# Autodesk Inventor assembly: mobile_robot_car_motor230
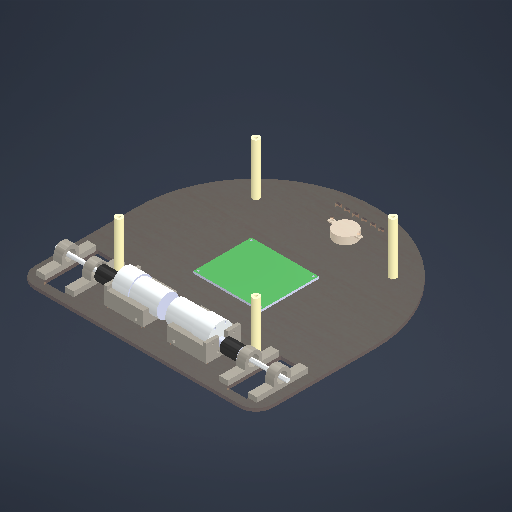
[picture p0: Inventor's stored thumbnail of the model, 512x512]
Saved by Autodesk Inventor 2026 (Build 300175050, 175E)
## iProperties
Created: 2025-06-05
Part Number: mobile_robot_car_motor230
Document SubType Name: Assembly
Designer: satom
Author: satom
## Documents named in this file (11)
- C:\Users\satom\Desktop\Robot\CAD\Inventor\mobile_robot_car_motor230.iam
- C:\Users\satom\Desktop\Robot\CAD\Inventor\C - Chassis\layer1_new_motor2.ipt
- C:\Users\satom\Desktop\Robot\CAD\Inventor\solidworks\D - DriveTrain\motor_FIT0403_122rpm\motor_FIT0403_122rpm\motor_FIT0403_122rpm.ipt
- C:\Users\satom\Desktop\Robot\CAD\Inventor\solidworks\D - DriveTrain\motor_holder_FIT0403_122rpm\motor_holder_FIT0403_122rpm\motor_holder_FIT0403_122rpm.ipt
- C:\Users\satom\Desktop\Robot\CAD\Inventor\solidworks\D - DriveTrain\wheel_bearing_FIT0403_122rpm\wheel_bearing_FIT0403_122rpm\wheel_bearing_FIT0403_122rpm.ipt
- C:\Users\satom\Desktop\Robot\CAD\Inventor\solidworks\D - DriveTrain\wheel_bearing\wheel_bearing\wheel_bearing.ipt
- C:\Users\satom\Desktop\Robot\CAD\Inventor\solidworks\D - DriveTrain\shaft_coupler 6 mm\shaft_coupler 6 mm\shaft_coupler 6 mm.ipt
- C:\Users\satom\Desktop\Robot\CAD\Inventor\solidworks\D - DriveTrain\drive_shaft\drive_shaft\drive_shaft.ipt
- C:\Users\satom\Desktop\Robot\CAD\Inventor\C - Chassis\3inch_standoff.ipt
- C:\Users\satom\Desktop\Robot\CAD\Inventor\solidworks\E - Electronics\Main Board\Main Board\Main Board.ipt
- C:\Users\satom\Desktop\Robot\CAD\Inventor\solidworks\D - DriveTrain\ball_caster\ball_caster\ball_caster.ipt
## Components (19 placed, 10 different names)
1. layer1_new_motor2:1 — Mate:1, Mate:2, Mate:9, Mate:10, Mate:11, Mate:12, Mate:13, Mate:14, Mate:15, Mate:16, Mate:17, Mate:18, Mate:19, Mate:20, Mate:21, Mate:22, Mate:23, Mate:24, Mate:25, Mate:26, Mate:35, Mate:36, Mate:37, Mate:38, Mate:39, Mate:40, Mate:41, Mate:42, Mate:43, Mate:44, Mate:45, Mate:46, Mate:47, Mate:48
2. motor_FIT0403_122rpm:1 — Mate:4, Mate:6, Mate:8, Mate:28, Mate:29
3. motor_FIT0403_122rpm:2 — Mate:3, Mate:5, Mate:7, Mate:27, Mate:30
4. motor_holder_FIT0403_122rpm:1 — Mate:2, Mate:4, Mate:6, Mate:8, Mate:12, Mate:13, Mate:14
5. motor_holder_FIT0403_122rpm:2 — Mate:1, Mate:3, Mate:5, Mate:7, Mate:9, Mate:10, Mate:11
6. wheel_bearing_FIT0403_122rpm:1 — Mate:15, Mate:16, Mate:17
7. wheel_bearing_FIT0403_122rpm:2 — Mate:18, Mate:19, Mate:20
8. wheel_bearing:1 — Mate:21, Mate:25, Mate:26
9. wheel_bearing:2 — Mate:22, Mate:23, Mate:24
10. shaft_coupler 6 mm:1 — Mate:27, Mate:30, Mate:32, Mate:33
11. shaft_coupler 6 mm:2 — Mate:28, Mate:29, Mate:31, Mate:34
12. drive_shaft:1 — Mate:32, Mate:33
13. drive_shaft:2 — Mate:31, Mate:34
14. 3inch_standoff:1 — Mate:36, Mate:37
15. 3inch_standoff:2 — Mate:35, Mate:38
16. Main Board:1 — Mate:39, Mate:40, Mate:41
17. ball_caster:1 — Mate:42, Mate:43, Mate:44
18. 3inch_standoff:3 — Mate:46, Mate:47
19. 3inch_standoff:4 — Mate:45, Mate:48
## Relationships (48: Mate 48)
- Mate:1: layer1_new_motor2:1 ↔ motor_holder_FIT0403_122rpm:2
- Mate:2: layer1_new_motor2:1 ↔ motor_holder_FIT0403_122rpm:1
- Mate:3: motor_FIT0403_122rpm:2 ↔ motor_holder_FIT0403_122rpm:2
- Mate:4: motor_FIT0403_122rpm:1 ↔ motor_holder_FIT0403_122rpm:1
- Mate:5: motor_FIT0403_122rpm:2 ↔ motor_holder_FIT0403_122rpm:2
- Mate:6: motor_FIT0403_122rpm:1 ↔ motor_holder_FIT0403_122rpm:1
- Mate:7: motor_FIT0403_122rpm:2 ↔ motor_holder_FIT0403_122rpm:2
- Mate:8: motor_FIT0403_122rpm:1 ↔ motor_holder_FIT0403_122rpm:1
- Mate:9: layer1_new_motor2:1 ↔ motor_holder_FIT0403_122rpm:2
- Mate:10: layer1_new_motor2:1 ↔ motor_holder_FIT0403_122rpm:2
- Mate:11: layer1_new_motor2:1 ↔ motor_holder_FIT0403_122rpm:2
- Mate:12: layer1_new_motor2:1 ↔ motor_holder_FIT0403_122rpm:1
- Mate:13: layer1_new_motor2:1 ↔ motor_holder_FIT0403_122rpm:1
- Mate:14: layer1_new_motor2:1 ↔ motor_holder_FIT0403_122rpm:1
- Mate:15: layer1_new_motor2:1 ↔ wheel_bearing_FIT0403_122rpm:1
- Mate:16: layer1_new_motor2:1 ↔ wheel_bearing_FIT0403_122rpm:1
- Mate:17: layer1_new_motor2:1 ↔ wheel_bearing_FIT0403_122rpm:1
- Mate:18: layer1_new_motor2:1 ↔ wheel_bearing_FIT0403_122rpm:2
- Mate:19: layer1_new_motor2:1 ↔ wheel_bearing_FIT0403_122rpm:2
- Mate:20: layer1_new_motor2:1 ↔ wheel_bearing_FIT0403_122rpm:2
- Mate:21: layer1_new_motor2:1 ↔ wheel_bearing:1
- Mate:22: layer1_new_motor2:1 ↔ wheel_bearing:2
- Mate:23: layer1_new_motor2:1 ↔ wheel_bearing:2
- Mate:24: layer1_new_motor2:1 ↔ wheel_bearing:2
- Mate:25: layer1_new_motor2:1 ↔ wheel_bearing:1
- Mate:26: layer1_new_motor2:1 ↔ wheel_bearing:1
- Mate:27: motor_FIT0403_122rpm:2 ↔ shaft_coupler 6 mm:1
- Mate:28: motor_FIT0403_122rpm:1 ↔ shaft_coupler 6 mm:2
- Mate:29: motor_FIT0403_122rpm:1 ↔ shaft_coupler 6 mm:2
- Mate:30: motor_FIT0403_122rpm:2 ↔ shaft_coupler 6 mm:1
- Mate:31: shaft_coupler 6 mm:2 ↔ drive_shaft:2
- Mate:32: shaft_coupler 6 mm:1 ↔ drive_shaft:1
- Mate:33: shaft_coupler 6 mm:1 ↔ drive_shaft:1
- Mate:34: shaft_coupler 6 mm:2 ↔ drive_shaft:2
- Mate:35: layer1_new_motor2:1 ↔ 3inch_standoff:2
- Mate:36: layer1_new_motor2:1 ↔ 3inch_standoff:1
- Mate:37: layer1_new_motor2:1 ↔ 3inch_standoff:1
- Mate:38: layer1_new_motor2:1 ↔ 3inch_standoff:2
- Mate:39: layer1_new_motor2:1 ↔ Main Board:1
- Mate:40: layer1_new_motor2:1 ↔ Main Board:1
- Mate:41: layer1_new_motor2:1 ↔ Main Board:1
- Mate:42: layer1_new_motor2:1 ↔ ball_caster:1
- Mate:43: layer1_new_motor2:1 ↔ ball_caster:1
- Mate:44: layer1_new_motor2:1 ↔ ball_caster:1
- Mate:45: layer1_new_motor2:1 ↔ 3inch_standoff:4
- Mate:46: layer1_new_motor2:1 ↔ 3inch_standoff:3
- Mate:47: layer1_new_motor2:1 ↔ 3inch_standoff:3
- Mate:48: layer1_new_motor2:1 ↔ 3inch_standoff:4
